# Autodesk Inventor assembly: GearAssembly
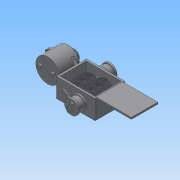
[picture p0: Inventor's stored thumbnail of the model, 180x180]
Saved by Autodesk Inventor 2015 (Build 190159000, 159)
## iProperties
Created: 2014-08-31
Part Number: GearAssembly
Document SubType Name: Assembly
Designer: shohei
Author: shohei
## Documents named in this file (11)
- C:\Users\shohei\Documents\Inventor\FufuPounderGeared\GearAssembly_rev1.iam
- C:\Users\shohei\Documents\Inventor\FufuPounderGeared\alternator.ipt
- C:\Users\shohei\Documents\Inventor\FufuPounderGeared\schaft1.ipt
- C:\Users\shohei\Documents\Inventor\FufuPounderGeared\Spur Gears1.iam
- C:\Users\shohei\Documents\Inventor\FufuPounderGeared\Spur Gears2.iam
- C:\Users\shohei\Documents\Inventor\FufuPounderGeared\shaft_cover.ipt
- C:\Users\shohei\Documents\Inventor\FufuPounderGeared\gearSupport.ipt
- C:\Users\shohei\Documents\Inventor\FufuPounderGeared\boxsupport.ipt
- C:\Users\shohei\Documents\Inventor\FufuPounderGeared\boxsupport2.ipt
- C:\Users\shohei\Documents\Inventor\FufuPounderGeared\drivepulleyAssembly.iam
- C:\Users\shohei\Documents\Inventor\FufuPounderGeared\pulleyFlange.ipt
## Components (27 placed, 9 different names)
1. alternator:1 — Angle:11
2. schaft1:1 — Mate:2, Mate:4, Rotational:8, Rigid:2, Cylindrical:1, Rigid:3, Rigid:4, Rotational:19, Rigid:6
3. schaft1:2 — Mate:4, Mate:6, Rigid:1, Rotational:20, Rotational:28, Rigid:5, Angle:10
4. Spur Gears:1 [sub-assembly] — Rotational:8, Angle:4, Angle:7, Rotational:18, Rotation:1
5. Spur Gears:3 [sub-assembly] — Angle:2, Rotational:25, Rotation:1
6. Spur Gears:4 [sub-assembly] — Angle:3, Rotational:17, Mate:16, Rotational:26, Rotation:3
7. Spur Gears:5 [sub-assembly] — Angle:2, Rotational:24, Rotational:25, Rotation:2
8. Spur Gears:6 [sub-assembly] — Rotational:17, Angle:6, Mate:22, Rotational:27, Rotation:4
9. Spur Gears:7 [sub-assembly] — Angle:3, Rotational:18, Mate:16, Rotational:26, Rotation:2
10. Spur Gears:8 [sub-assembly] — Angle:6, Mate:22, Rotational:27, Rotation:5
11. Spur Gears:9 [sub-assembly] — Angle:5, Rotational:22, Mate:21, Rotational:23, Rotation:4
12. Spur Gears:10 [sub-assembly] — Angle:5, Mate:21, Rotational:23, Rotational:24, Rotation:3
13. shaft_cover:1 — Mate:13, Flush:8, Flush:9, Cylindrical:1, Mate:20, Rotational:28, Angle:11, Mate:23, Flush:12
14. Spur Gears:11 [sub-assembly] — Angle:8, Rotational:20, Rotational:21, Rotational:22, Rotation:5, Angle:9
15. shaft_cover:2 — Flush:10, Flush:11, Mate:17, Mate:18
16. gearSupport:1 — Angle:7, Rotational:19, Rigid:6
17. gearSupport:2 — Angle:8, Rotational:21, Angle:10
18. boxsupport:1 — Flush:5, Flush:7, Mate:12, Flush:11, Mate:18, Mate:19
19. boxsupport:2 — Mate:23, Flush:12
20. boxsupport2:1 — Flush:7, Mate:12, Mate:20
21. boxsupport2:2 — Flush:5, Mate:13, Flush:8, Flush:9, Flush:10, Mate:17, Mate:19
22. drivepulleyAssembly:1 [sub-assembly] — Rigid:2
23. drivepulleyAssembly:2 [sub-assembly] — Rigid:1, Mate:14, Mate:15
24. pulleyFlange:1 — Mate:14, Mate:15
25. pulleyFlange:2 — Rigid:4
26. pulleyFlange:3 — Rigid:3
27. pulleyFlange:4 — Rigid:5
## Relationships (57: Mate 15, RevoluteJoint 13, Angle 10, Flush 7, WeldJoint 6, RelateRotation 5, CylindricalJoint 1)
- Mate:2: schaft1:1
- Mate:4 (70 mm): schaft1:1 ↔ schaft1:2
- Mate:6: schaft1:2
- Angle:2 (0 deg): Spur Gears:3 ↔ Spur Gears:5
- Rotational:8 [RevoluteJoint] (-105 mm): schaft1:1 ↔ Spur Gears:1
- Angle:3 (0 deg): Spur Gears:4 ↔ Spur Gears:7
- Angle:4 (300 deg): Spur Gears:1
- Angle:5 (0 deg): Spur Gears:9 ↔ Spur Gears:10
- Rotational:17 [RevoluteJoint]: Spur Gears:4 ↔ Spur Gears:6
- Angle:6 (0 deg): Spur Gears:6 ↔ Spur Gears:8
- Angle:7 (0 deg): Spur Gears:1 ↔ gearSupport:1
- Angle:8 (0 deg): Spur Gears:11 ↔ gearSupport:2
- Flush:5: boxsupport:1 ↔ boxsupport2:2
- Flush:7: boxsupport:1 ↔ boxsupport2:1
- Rigid:1 [WeldJoint]: schaft1:2 ↔ drivepulleyAssembly:2
- Rigid:2 [WeldJoint] (-10 mm): schaft1:1 ↔ drivepulleyAssembly:1
- Mate:12: boxsupport:1 ↔ boxsupport2:1
- Mate:13: shaft_cover:1 ↔ boxsupport2:2
- Flush:8: shaft_cover:1 ↔ boxsupport2:2
- Flush:9: shaft_cover:1 ↔ boxsupport2:2
- Flush:10: shaft_cover:2 ↔ boxsupport2:2
- Flush:11: shaft_cover:2 ↔ boxsupport:1
- Cylindrical:1: schaft1:1 ↔ shaft_cover:1
- Mate:14: drivepulleyAssembly:2 ↔ pulleyFlange:1
- Mate:15: drivepulleyAssembly:2 ↔ pulleyFlange:1
- Rigid:3 [WeldJoint]: schaft1:1 ↔ pulleyFlange:3
- Rigid:4 [WeldJoint]: schaft1:1 ↔ pulleyFlange:2
- Rotational:19 [RevoluteJoint] (-15 mm): schaft1:1 ↔ gearSupport:1
- Rotational:18 [RevoluteJoint]: Spur Gears:1 ↔ Spur Gears:7
- Mate:16: Spur Gears:4 ↔ Spur Gears:7
- Mate:17: shaft_cover:2 ↔ boxsupport2:2
- Mate:18: shaft_cover:2 ↔ boxsupport:1
- Mate:19: boxsupport:1 ↔ boxsupport2:2
- Mate:20: shaft_cover:1 ↔ boxsupport2:1
- Rotational:20 [RevoluteJoint] (30 mm): schaft1:2 ↔ Spur Gears:11
- Rotational:21 [RevoluteJoint]: Spur Gears:11 ↔ gearSupport:2
- Rotational:22 [RevoluteJoint]: Spur Gears:9 ↔ Spur Gears:11
- Mate:21: Spur Gears:9 ↔ Spur Gears:10
- Rotational:23 [RevoluteJoint]: Spur Gears:9 ↔ Spur Gears:10
- Rotational:24 [RevoluteJoint]: Spur Gears:5 ↔ Spur Gears:10
- Rotational:25 [RevoluteJoint]: Spur Gears:3 ↔ Spur Gears:5
- Rotational:26 [RevoluteJoint]: Spur Gears:4 ↔ Spur Gears:7
- Mate:22: Spur Gears:6 ↔ Spur Gears:8
- Rotational:27 [RevoluteJoint]: Spur Gears:6 ↔ Spur Gears:8
- Rotation:1 [RelateRotation] (1.6 ul): Spur Gears:1 ↔ Spur Gears:3
- Rotation:2 [RelateRotation] (1.6 ul): Spur Gears:5 ↔ Spur Gears:7
- Rotational:28 [RevoluteJoint] (-30 mm): schaft1:2 ↔ shaft_cover:1
- Rigid:5 [WeldJoint]: schaft1:2 ↔ pulleyFlange:4
- Rotation:3 [RelateRotation] (1.6 ul): Spur Gears:4 ↔ Spur Gears:10
- Rotation:4 [RelateRotation] (1.6 ul): Spur Gears:6 ↔ Spur Gears:9
- Rotation:5 [RelateRotation] (1.6 ul): Spur Gears:8 ↔ Spur Gears:11
- Rigid:6 [WeldJoint] (-25 mm): schaft1:1 ↔ gearSupport:1
- Angle:9 (0 deg): Spur Gears:11
- Angle:10 (0 deg): schaft1:2 ↔ gearSupport:2
- Angle:11 (180 deg): alternator:1 ↔ shaft_cover:1
- Mate:23: shaft_cover:1 ↔ boxsupport:2
- Flush:12: shaft_cover:1 ↔ boxsupport:2
